# Autodesk Inventor assembly: Roboter3_neu
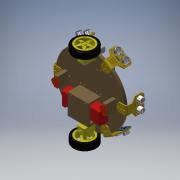
[picture p0: Inventor's stored thumbnail of the model, 180x180]
Saved by Autodesk Inventor 2017 SP1 (Build 210196100, 196)
## iProperties
Part Number: Roboter3_neu
Material: Generisch
Document SubType Name: Assembly
Designer: Alex
Author: Alex
## Documents named in this file (14)
- E:\Users\Alex\Documents\Inventor\Roboter\Finish\Roboter.iam
- E:\Users\Alex\Documents\Inventor\Roboter\Finish\Platte3_neu.ipt
- E:\Users\Alex\Documents\Inventor\Roboter\Finish\AkkuHaltSeitenWand.ipt
- E:\Users\Alex\Documents\Inventor\Roboter\Finish\AkkuHaltBoden.ipt
- E:\Users\Alex\Documents\Inventor\Roboter\Finish\Akku_3S_2700.ipt
- E:\Users\Alex\Documents\Inventor\Roboter\Finish\KugelRadStützen.ipt
- E:\Users\Alex\Documents\Inventor\Motor_Driver\Motor_Driver.iam
- E:\Users\Alex\Documents\Inventor\RaspberryPi\Raspberry Pi 3.iam
- E:\Users\Alex\Documents\Inventor\Roboter\Finish\PCB_4x6.ipt
- E:\Users\Alex\Documents\Inventor\Roboter\Finish\Motor_plus_Rad.iam
- E:\Users\Alex\Documents\Inventor\Roboter\Finish\KugelradAdapter.ipt
- E:\Users\Alex\Documents\Inventor\Roboter\Finish\Gruppe.iam
- E:\Users\Alex\Documents\Inventor\Roboter\Finish\arduino MEGA2650.iam
- E:\Users\Alex\Documents\Inventor\Roboter\Finish\LM2596.iam
## Components (22 placed, 13 different names)
1. Platte3_neu:1 — Passend:1, Passend:2, Passend:3, Passend:4, Passend:5, Passend:6, Passend:7, Passend:8, Passend:9, Passend:10, Passend:11, Passend:12, Passend:22, Passend:23, Passend:24, Passend:25, Passend:26, Passend:27, Passend:28, Passend:29, Passend:30, Passend:33, Passend:34, Passend:35, Passend:36, Passend:37, Passend:38, Passend:39, Passend:40, Passend:41, Passend:42, Passend:43, Passend:44, Passend:45, Passend:46, Passend:47, Passend:48, Passend:49, Passend:50, Passend:51, Passend:52, Passend:53, Passend:54, Passend:55, Passend:56, Passend:57, Passend:58, Passend:59, Passend:60, Passend:61
2. AkkuHaltSeitenWand:1 — Passend:10, Passend:11, Passend:12, Passend:14, Passend:15
3. AkkuHaltSeitenWand:2 — Passend:7, Passend:8, Passend:9, Passend:13, Passend:32
4. AkkuHaltBoden:1 — Passend:13, Passend:14, Passend:15, Passend:31
5. Akku_3S_2700:1 — Passend:31, Passend:32
6. KugelRadStützen:1 — Passend:4, Passend:5, Passend:6, Passend:19, Passend:20, Passend:21
7. KugelRadStützen:2 — Passend:1, Passend:2, Passend:3, Passend:16, Passend:17, Passend:18
8. Motor_Driver:1 [sub-assembly] — Passend:33, Passend:34, Passend:35
9. Raspberry Pi 3:1 [sub-assembly] — Passend:28, Passend:29, Passend:30
10. PCB_4x6:1 — Passend:36, Passend:37, Passend:38, Fluchtend:1
11. Motor_plus_Rad:1 [sub-assembly] — Passend:22, Passend:23, Passend:24
12. Motor_plus_Rad:2 [sub-assembly] — Passend:25, Passend:26, Passend:27
13. KugelradAdapter:1 — Passend:16, Passend:17, Passend:18
14. KugelradAdapter:2 — Passend:19, Passend:20, Passend:21
15. Gruppe:1 [sub-assembly] — Passend:51, Passend:52, Passend:53
16. Gruppe:2 [sub-assembly] — Passend:54, Passend:55, Passend:56
17. Gruppe:3 [sub-assembly] — Passend:39, Passend:40, Passend:41
18. Gruppe:4 [sub-assembly] — Passend:42, Passend:43, Passend:44
19. Gruppe:5 [sub-assembly] — Passend:45, Passend:46, Passend:47
20. Gruppe:6 [sub-assembly] — Passend:48, Passend:49, Passend:50
21. arduino MEGA2650:1 [sub-assembly] — Passend:57, Passend:58, Passend:59
22. LM2596:1 [sub-assembly] — Fluchtend:1, Passend:60, Passend:61
## Relationships (62: Mate 61, Flush 1)
- Passend:1 [Mate]: Platte3_neu:1 ↔ KugelRadStützen:2
- Passend:2 [Mate]: Platte3_neu:1 ↔ KugelRadStützen:2
- Passend:3 [Mate]: Platte3_neu:1 ↔ KugelRadStützen:2
- Passend:4 [Mate]: Platte3_neu:1 ↔ KugelRadStützen:1
- Passend:5 [Mate]: Platte3_neu:1 ↔ KugelRadStützen:1
- Passend:6 [Mate]: Platte3_neu:1 ↔ KugelRadStützen:1
- Passend:7 [Mate]: Platte3_neu:1 ↔ AkkuHaltSeitenWand:2
- Passend:8 [Mate]: Platte3_neu:1 ↔ AkkuHaltSeitenWand:2
- Passend:9 [Mate]: Platte3_neu:1 ↔ AkkuHaltSeitenWand:2
- Passend:10 [Mate]: Platte3_neu:1 ↔ AkkuHaltSeitenWand:1
- Passend:11 [Mate]: Platte3_neu:1 ↔ AkkuHaltSeitenWand:1
- Passend:12 [Mate]: Platte3_neu:1 ↔ AkkuHaltSeitenWand:1
- Passend:13 [Mate]: AkkuHaltSeitenWand:2 ↔ AkkuHaltBoden:1
- Passend:14 [Mate]: AkkuHaltSeitenWand:1 ↔ AkkuHaltBoden:1
- Passend:15 [Mate]: AkkuHaltSeitenWand:1 ↔ AkkuHaltBoden:1
- Passend:16 [Mate]: KugelRadStützen:2 ↔ KugelradAdapter:1
- Passend:17 [Mate]: KugelRadStützen:2 ↔ KugelradAdapter:1
- Passend:18 [Mate]: KugelRadStützen:2 ↔ KugelradAdapter:1
- Passend:19 [Mate]: KugelRadStützen:1 ↔ KugelradAdapter:2
- Passend:20 [Mate]: KugelRadStützen:1 ↔ KugelradAdapter:2
- Passend:21 [Mate]: KugelRadStützen:1 ↔ KugelradAdapter:2
- Passend:22 [Mate]: Platte3_neu:1 ↔ Motor_plus_Rad:1
- Passend:23 [Mate]: Platte3_neu:1 ↔ Motor_plus_Rad:1
- Passend:24 [Mate]: Platte3_neu:1 ↔ Motor_plus_Rad:1
- Passend:25 [Mate]: Platte3_neu:1 ↔ Motor_plus_Rad:2
- Passend:26 [Mate]: Platte3_neu:1 ↔ Motor_plus_Rad:2
- Passend:27 [Mate]: Platte3_neu:1 ↔ Motor_plus_Rad:2
- Passend:28 [Mate]: Platte3_neu:1 ↔ Raspberry Pi 3:1
- Passend:29 [Mate] (5 mm): Platte3_neu:1 ↔ Raspberry Pi 3:1
- Passend:30 [Mate]: Platte3_neu:1 ↔ Raspberry Pi 3:1
- Passend:31 [Mate]: AkkuHaltBoden:1 ↔ Akku_3S_2700:1
- Passend:32 [Mate] (5 mm): AkkuHaltSeitenWand:2 ↔ Akku_3S_2700:1
- Passend:33 [Mate]: Platte3_neu:1 ↔ Motor_Driver:1
- Passend:34 [Mate]: Platte3_neu:1 ↔ Motor_Driver:1
- Passend:35 [Mate] (5 mm): Platte3_neu:1 ↔ Motor_Driver:1
- Passend:36 [Mate]: Platte3_neu:1 ↔ PCB_4x6:1
- Passend:37 [Mate]: Platte3_neu:1 ↔ PCB_4x6:1
- Passend:38 [Mate] (5 mm): Platte3_neu:1 ↔ PCB_4x6:1
- Passend:39 [Mate]: Platte3_neu:1 ↔ Gruppe:3
- Passend:40 [Mate]: Platte3_neu:1 ↔ Gruppe:3
- Passend:41 [Mate]: Platte3_neu:1 ↔ Gruppe:3
- Passend:42 [Mate]: Platte3_neu:1 ↔ Gruppe:4
- Passend:43 [Mate]: Platte3_neu:1 ↔ Gruppe:4
- Passend:44 [Mate]: Platte3_neu:1 ↔ Gruppe:4
- Passend:45 [Mate]: Platte3_neu:1 ↔ Gruppe:5
- Passend:46 [Mate]: Platte3_neu:1 ↔ Gruppe:5
- Passend:47 [Mate]: Platte3_neu:1 ↔ Gruppe:5
- Passend:48 [Mate]: Platte3_neu:1 ↔ Gruppe:6
- Passend:49 [Mate]: Platte3_neu:1 ↔ Gruppe:6
- Passend:50 [Mate]: Platte3_neu:1 ↔ Gruppe:6
- Passend:51 [Mate]: Platte3_neu:1 ↔ Gruppe:1
- Passend:52 [Mate]: Platte3_neu:1 ↔ Gruppe:1
- Passend:53 [Mate]: Platte3_neu:1 ↔ Gruppe:1
- Passend:54 [Mate]: Platte3_neu:1 ↔ Gruppe:2
- Passend:55 [Mate]: Platte3_neu:1 ↔ Gruppe:2
- Passend:56 [Mate]: Platte3_neu:1 ↔ Gruppe:2
- Passend:57 [Mate]: Platte3_neu:1 ↔ arduino MEGA2650:1
- Passend:58 [Mate]: Platte3_neu:1 ↔ arduino MEGA2650:1
- Passend:59 [Mate] (5 mm): Platte3_neu:1 ↔ arduino MEGA2650:1
- Fluchtend:1 [Flush]: PCB_4x6:1 ↔ LM2596:1
- Passend:60 [Mate]: Platte3_neu:1 ↔ LM2596:1
- Passend:61 [Mate]: Platte3_neu:1 ↔ LM2596:1
